# Autodesk Inventor assembly: SmallCGearN'MLock
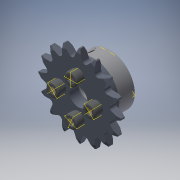
[picture p0: Inventor's stored thumbnail of the model, 180x180]
Saved by Autodesk Inventor 2016 (Build 200138000, 138)
## iProperties
Created: 2015-09-01
Part Number: SmallCGearN'MLock
Document SubType Name: Assembly
Designer: Tim
Author: Tim
## Documents named in this file (4)
- C:\Users\Tim\Documents\GitHub\phi_robotics\3d-models\FTC_Tetrix_KOP_Block_Party\Tim Bloot Designs\SmallCGearN'MLock.iam
- C:\Users\Tim\Documents\GitHub\phi_robotics\3d-models\FTC_Tetrix_KOP_Block_Party\Tetrix_Kit_FTC\Autodesk Inventor Files\tetrix_chain_gear-16t.ipt
- C:\Users\Tim\Documents\GitHub\phi_robotics\3d-models\FTC_Tetrix_KOP_Block_Party\Tetrix_Kit_FTC\Autodesk Inventor Files\tetrix_maxle_lock.iam
- C:\Users\Tim\Documents\GitHub\phi_robotics\3d-models\FTC_Tetrix_KOP_Block_Party\Tetrix_Kit_FTC\Autodesk Inventor Files\tetrix_screw.ipt
## Components (6 placed, 3 different names)
1. tetrix_chain_gear-16t:1 — Rigid:1, Rigid:2, Rigid:3, Rigid:4, Rigid:5
2. tetrix_maxle_lock:1 [sub-assembly] — Rigid:1
3. tetrix_screw:1 — Rigid:2
4. tetrix_screw:2 — Rigid:3
5. tetrix_screw:3 — Rigid:4
6. tetrix_screw:4 — Rigid:5
## Relationships (5: WeldJoint 5)
- Rigid:1 [WeldJoint]: tetrix_chain_gear-16t:1 ↔ tetrix_maxle_lock:1
- Rigid:2 [WeldJoint]: tetrix_chain_gear-16t:1 ↔ tetrix_screw:1
- Rigid:3 [WeldJoint]: tetrix_chain_gear-16t:1 ↔ tetrix_screw:2
- Rigid:4 [WeldJoint]: tetrix_chain_gear-16t:1 ↔ tetrix_screw:3
- Rigid:5 [WeldJoint]: tetrix_chain_gear-16t:1 ↔ tetrix_screw:4
